# Autodesk Inventor assembly: USB-TypeB-Female-PanelMount
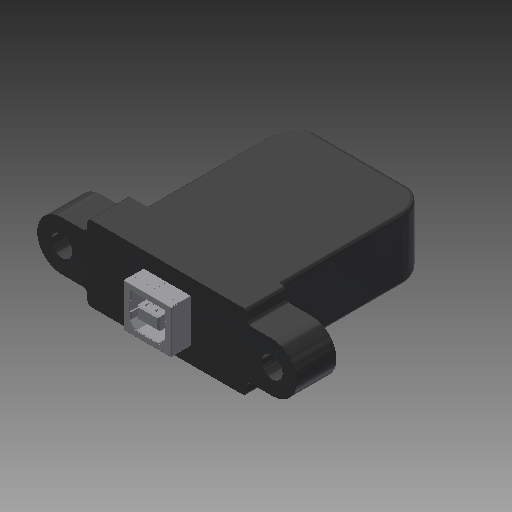
[picture p0: Inventor's stored thumbnail of the model, 512x512]
Saved by Autodesk Inventor 2017 (Build 210142000, 142)
## iProperties
Created: 2020-10-05
Part Number: USB-TypeB-Female-PanelMount
Document SubType Name: Assembly
Designer: Joe Ferner
Author: Joe Ferner
## Documents named in this file (3)
- C:\dev\raspberry-pi-ir-hat\models3d\USB-TypeB-Female-PanelMount\USB-TypeB-Female-PanelMount.iam
- C:\dev\raspberry-pi-ir-hat\models3d\USB-TypeB-Female-PanelMount\USB-TypeB-Female.ipt
- C:\dev\raspberry-pi-ir-hat\models3d\USB-TypeB-Female-PanelMount\panel-mount.ipt
## Components (2 placed, 2 different names)
1. USB-TypeB-Female:1 — Mate:1, Mate:2, Flush:1
2. panel-mount:1 — Mate:1, Mate:2, Flush:1
## Relationships (3: Mate 2, Flush 1)
- Mate:1: USB-TypeB-Female:1 ↔ panel-mount:1
- Mate:2: USB-TypeB-Female:1 ↔ panel-mount:1
- Flush:1 (-5 mm): USB-TypeB-Female:1 ↔ panel-mount:1
